# Autodesk Inventor assembly: Suporte Superior
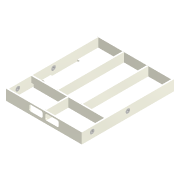
[picture p0: Inventor's stored thumbnail of the model, 180x180]
Saved by Autodesk Inventor 2020 (Build 240168000, 168)
## iProperties
Created: 2021-09-21
Part Number: Suporte Superior
Document SubType Name: Assembly
Designer: pablo
Author: pablo
## Documents named in this file (9)
- C:\Google Drive\Pablo Arquivos\Projetos\Utilidades Domesticas\Talheres\Suporte Superior.iam
- C:\Google Drive\Pablo Arquivos\Projetos\Utilidades Domesticas\Talheres\Divisória-22cm.ipt
- C:\Google Drive\Pablo Arquivos\Projetos\Utilidades Domesticas\Talheres\Third\AIS2019\SKF_619_6-2Z.iam
- C:\Google Drive\Pablo Arquivos\Projetos\Utilidades Domesticas\Talheres\Divisória-25cm.ipt
- C:\Google Drive\Pablo Arquivos\Projetos\Utilidades Domesticas\Talheres\Divisória-24cm.ipt
- C:\Google Drive\Pablo Arquivos\Projetos\Utilidades Domesticas\Talheres\Divisória-7,5cm.ipt
- C:\Google Drive\Pablo Arquivos\Projetos\Utilidades Domesticas\Talheres\Divisória-25cm Frontal.ipt
- C:\Google Drive\Pablo Arquivos\Projetos\Utilidades Domesticas\Talheres\Divisória-30cm c rolamento - superior.ipt
- C:\Google Drive\Pablo Arquivos\Projetos\Utilidades Domesticas\Talheres\Base Superior.ipt
## Components (13 placed, 8 different names)
1. Divisória-22cm:1 — Mate:29, Mate:30
2. Divisória-22cm:2 — Mate:31, Mate:32
3. SKF_619_6-2Z:1 [sub-assembly] — Mate:43
4. SKF_619_6-2Z:2 [sub-assembly] — Mate:42
5. SKF_619_6-2Z:3 [sub-assembly] — Mate:36
6. SKF_619_6-2Z:4 [sub-assembly] — Mate:37
7. Divisória-25cm:2 — Mate:40, Mate:41
8. Divisória-24cm:1 — Mate:44, Mate:45, Mate:46
9. Divisória-7,5cm:1 — Mate:33, Mate:34, Mate:35, Mate:45
10. Divisória-25cm Frontal:1 — Mate:25, Mate:26, Mate:34
11. Divisória-30cm c rolamento - superior:1 — Mate:27, Mate:28, Mate:35, Mate:36, Mate:37
12. Base Superior:1 — Mate:25, Mate:26, Mate:27, Mate:28, Mate:29, Mate:30, Mate:31, Mate:32, Mate:33, Mate:38, Mate:39, Mate:40, Mate:41, Mate:44, Mate:46
13. Divisória-30cm c rolamento - superior:2 — Mate:38, Mate:39, Mate:42, Mate:43
## Relationships (22: Mate 22)
- Mate:25: Divisória-25cm Frontal:1 ↔ Base Superior:1
- Mate:26: Divisória-25cm Frontal:1 ↔ Base Superior:1
- Mate:27: Divisória-30cm c rolamento - superior:1 ↔ Base Superior:1
- Mate:28: Divisória-30cm c rolamento - superior:1 ↔ Base Superior:1
- Mate:29: Divisória-22cm:1 ↔ Base Superior:1
- Mate:30: Divisória-22cm:1 ↔ Base Superior:1
- Mate:31: Divisória-22cm:2 ↔ Base Superior:1
- Mate:32: Divisória-22cm:2 ↔ Base Superior:1
- Mate:33: Divisória-7,5cm:1 ↔ Base Superior:1
- Mate:34: Divisória-7,5cm:1 ↔ Divisória-25cm Frontal:1
- Mate:35 (120 mm): Divisória-7,5cm:1 ↔ Divisória-30cm c rolamento - superior:1
- Mate:36: SKF_619_6-2Z:3 ↔ Divisória-30cm c rolamento - superior:1
- Mate:37: SKF_619_6-2Z:4 ↔ Divisória-30cm c rolamento - superior:1
- Mate:38: Base Superior:1 ↔ Divisória-30cm c rolamento - superior:2
- Mate:39: Base Superior:1 ↔ Divisória-30cm c rolamento - superior:2
- Mate:40: Divisória-25cm:2 ↔ Base Superior:1
- Mate:41: Divisória-25cm:2 ↔ Base Superior:1
- Mate:42: SKF_619_6-2Z:2 ↔ Divisória-30cm c rolamento - superior:2
- Mate:43: SKF_619_6-2Z:1 ↔ Divisória-30cm c rolamento - superior:2
- Mate:44: Divisória-24cm:1 ↔ Base Superior:1
- Mate:45: Divisória-24cm:1 ↔ Divisória-7,5cm:1
- Mate:46: Divisória-24cm:1 ↔ Base Superior:1
